# Autodesk Inventor assembly: ESTAMP Post 683110
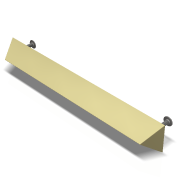
[picture p0: Inventor's stored thumbnail of the model, 180x180]
Saved by Autodesk Inventor 2024 (Build 280153000, 153)
## iProperties
RuleStatus: InUse
Created: 2023-02-20
Part Number: ESTAMP Post 683110
Document SubType Name: Assembly
Designer: sauliusd
Author: sauliusd
## Documents named in this file (5)
- C:\W4INV 2024 Design\PROJECTS\Samples\Commode\COM.iam Smart Hardware\ESTAMP Post 683110\ESTAMP Post 683110.iam
- C:\W4INV 2024 Design\PROJECTS\Samples\Commode\COM.iam Smart Hardware\ESTAMP Post 683110\ESTAMP Post 68311001.ipt
- C:\W4INV 2024 Design\PROJECTS\MODEL STATE LIBRARY COMPONENTS\Handles\ESTAMP Post 683.ipt
- C:\W4INV 2024 Design\PROJECTS\Samples\Commode\COM.iam Smart Hardware\ESTAMP Post 683110\ESTAMP Post 68311000.ipt
- C:\W4INV 2024 Design\LIBRARY\Handles\M4 Threated Screw.ipt
## Components (6 placed, 5 different names)
1. @Skeleton — Flush:1, Flush:2
2. ESTAMP Post 683 Handle — Flush:1, Flush:2, Insert:1, Insert:2, Flush:3
3. ESAMP Handle Hole_1 — Insert:1, Insert:3
4. ESAMP Handle Hole_2 — Insert:2, Insert:4
5. M4 Threated Screw:1 — Insert:3
6. M4 Threated Screw:2 — Insert:4
## Relationships (7: Insert 4, Flush 3)
- Flush:1: @Skeleton ↔ ESTAMP Post 683 Handle
- Flush:2: @Skeleton ↔ ESTAMP Post 683 Handle
- Insert:1: ESTAMP Post 683 Handle ↔ ESAMP Handle Hole_1
- Insert:2: ESTAMP Post 683 Handle ↔ ESAMP Handle Hole_2
- Insert:3: ESAMP Handle Hole_1 ↔ M4 Threated Screw:1
- Insert:4: ESAMP Handle Hole_2 ↔ M4 Threated Screw:2
- Flush:3: ESTAMP Post 683 Handle
## Named parameters: HandleLength = 213 mm, FacadeWidth = 918 mm, FacadeHeight = 177.5 mm, DistFromSide_X = 44 mm, DistFromSide_Y = 44 mm, FacadeThickness = 18 mm, Shift_X = 0 mm, Shift_Y = 0 mm
